# Autodesk Inventor assembly: 惯性筛筛网装配
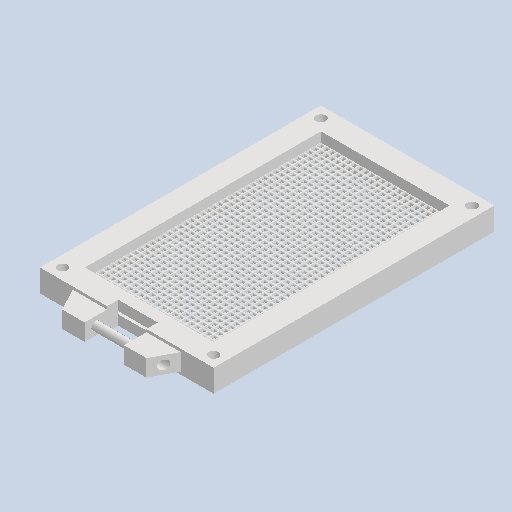
[picture p0: Inventor's stored thumbnail of the model, 512x512]
Saved by Autodesk Inventor 2022 (Build 260153000, 153)
## iProperties
Created: 2022-05-21
Part Number: 惯性筛筛网装配
Document SubType Name: Assembly
Designer: zhcne
Author: zhcne
## Documents named in this file (5)
- E:\Engineering_Development\SchoolProjects\2022_5_18_惯性筛_机电一体化课程设计\inertiascreen_curriculumdesign\3.Model\2.3D_Simulation\惯性筛筛网装配.iam
- E:\Engineering_Development\SchoolProjects\2022_5_18_惯性筛_机电一体化课程设计\inertiascreen_curriculumdesign\3.Model\2.3D_Simulation\Ipt\3.筛网\筛网上.ipt
- E:\Engineering_Development\SchoolProjects\2022_5_18_惯性筛_机电一体化课程设计\inertiascreen_curriculumdesign\3.Model\2.3D_Simulation\Ipt\3.筛网\筛网下.ipt
- E:\Engineering_Development\SchoolProjects\2022_5_18_惯性筛_机电一体化课程设计\inertiascreen_curriculumdesign\3.Model\2.3D_Simulation\Ipt\3.筛网\筛网.ipt
- E:\Engineering_Development\SchoolProjects\2022_5_18_惯性筛_机电一体化课程设计\inertiascreen_curriculumdesign\3.Model\2.3D_Simulation\Ipt\3.筛网\轴.ipt
## Components (4 placed, 4 different names)
1. 筛网上:1 — 配合:1, 配合:2, 配合:3, 配合:4, 表面齐平:1, 表面齐平:2, 配合:6
2. 筛网下:1 — 配合:1, 表面齐平:1, 表面齐平:2, 配合:5
3. 筛网:1 — 配合:2, 配合:3, 配合:4
4. 轴:1 — 配合:5, 配合:6
## Relationships (8: Mate 6, Flush 2)
- 配合:1 [Mate]: 筛网上:1 ↔ 筛网下:1
- 配合:2 [Mate] (0.5 mm): 筛网上:1 ↔ 筛网:1
- 配合:3 [Mate] (0.9 mm): 筛网上:1 ↔ 筛网:1
- 配合:4 [Mate] (1 mm): 筛网上:1 ↔ 筛网:1
- 表面齐平:1 [Flush]: 筛网上:1 ↔ 筛网下:1
- 表面齐平:2 [Flush]: 筛网上:1 ↔ 筛网下:1
- 配合:5 [Mate] (-3 mm): 筛网下:1 ↔ 轴:1
- 配合:6 [Mate]: 筛网上:1 ↔ 轴:1
